# Autodesk Inventor assembly: frame
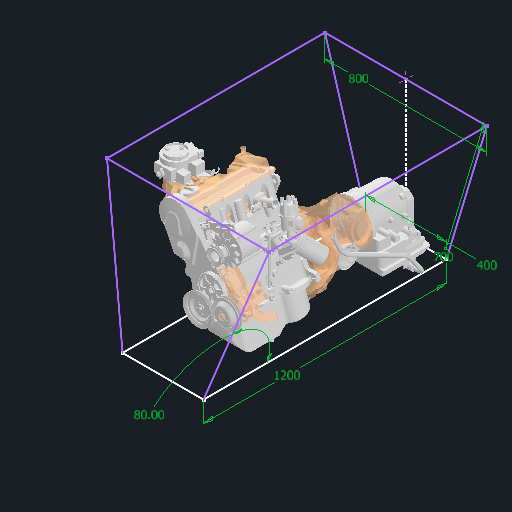
[picture p0: Inventor's stored thumbnail of the model, 512x512]
Saved by Autodesk Inventor 2025.3 (Build 293356000, 356)
## iProperties
Created: 2026-09-23
Part Number: frame
Document SubType Name: Assembly
Designer: VianaCC
Author: VianaCC
## Documents named in this file (3)
- C:\Users\vianacc\Documents\GitHub\utv_startup\products\utv\chassis\cad\draft\frame.iam
- C:\Users\vianacc\Documents\GitHub\utv_startup\products\utv\powertrain\cad\reference\motor-volkswagen-ap-1800-cc-de-1\Paulo R Conjunto MOTOR VW AP 1800 - 1998\Paulo R Conjunto MOTOR VW AP 1800 - 1998\Paulo R Con.iam
- C:\Users\vianacc\Documents\GitHub\utv_startup\products\utv\chassis\cad\draft\frame_skel.ipt
## Components (2 placed, 2 different names)
1. Paulo R Con:1 [sub-assembly] — Mate:1
2. frame_skel:1
## Relationships (1: Mate 1)
- Mate:1: Paulo R Con:1
